# Autodesk Inventor assembly: ForeArmAssembly
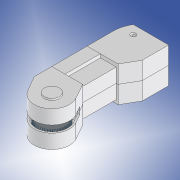
[picture p0: Inventor's stored thumbnail of the model, 180x180]
Saved by Autodesk Inventor 2017 (Build 210142000, 142)
## iProperties
Created: 2017-06-14
Part Number: ForeArmAssembly
Document SubType Name: Assembly
Designer: zallen
Author: zallen
## Documents named in this file (11)
- C:\Users\zallen\Documents\GitHub\cr-laundry-robot\src\Body\Arm Assembly\Bicep Assembly\BicepAssembly.iam
- C:\Users\zallen\Documents\GitHub\cr-laundry-robot\src\Body\Arm Assembly\Bicep Assembly\BA001.ipt
- C:\Users\zallen\Documents\GitHub\cr-laundry-robot\src\Body\Arm Assembly\Bicep Assembly\BA002.ipt
- C:\Users\zallen\Documents\GitHub\cr-laundry-robot\lib\Stepper Motor - NEMA 17\NEMA17.ipt
- C:\Users\zallen\Documents\GitHub\cr-laundry-robot\src\Body\Arm Assembly\Bicep Assembly\BA003.ipt
- C:\Users\zallen\Documents\GitHub\cr-laundry-robot\src\Body\Arm Assembly\Bicep Assembly\BA004.ipt
- C:\Users\zallen\Documents\GitHub\cr-laundry-robot\src\Body\Arm Assembly\Bicep Assembly\BA005.ipt
- C:\Users\zallen\Documents\GitHub\cr-laundry-robot\src\Body\Arm Assembly\Bicep Assembly\12 x 100mm Shaft.ipt
- C:\Users\zallen\Documents\GitHub\cr-laundry-robot\src\Body\Arm Assembly\Bicep Assembly\BicepAssembly\Design Accelerator\Spur Gears1.iam
- C:\Users\zallen\Documents\GitHub\cr-laundry-robot\lib\6201RS\6201RS.ipt
- C:\Users\zallen\Documents\GitHub\cr-laundry-robot\src\Body\Arm Assembly\Bicep Assembly\BA006.ipt
## Components (11 placed, 10 different names)
1. BA001:1 — Mate:1, Mate:3, Mate:4, Mate:5, Mate:8, Mate:12, Mate:18, Mate:41
2. BA002:1 — Mate:1, Mate:4, Mate:10, Mate:11
3. NEMA17:1 — Mate:3, Mate:5, Mate:18, Mate:40
4. BA003:1 — Mate:8, Mate:12, Mate:16, Mate:17
5. BA003:2 — Mate:10, Mate:11, Mate:13, Mate:14
6. BA004:1 — Mate:13, Mate:14, Mate:43, Mate:44
7. BA005:1 — Mate:16, Mate:17, Mate:19, Mate:20, Mate:33, Mate:38, Mate:42, Mate:43
8. 12 x 100mm Shaft:1 — Mate:19, Mate:20, Mate:35, Mate:44
9. Spur Gears:1 [sub-assembly] — Mate:33, Mate:35, Mate:36, Mate:37, Mate:38, Mate:42
10. 6201RS:1 — Mate:36, Mate:37
11. BA006:1 — Mate:40, Mate:41
## Relationships (25: Mate 25)
- Mate:1: BA001:1 ↔ BA002:1
- Mate:3: BA001:1 ↔ NEMA17:1
- Mate:4: BA001:1 ↔ BA002:1
- Mate:5: BA001:1 ↔ NEMA17:1
- Mate:8: BA001:1 ↔ BA003:1
- Mate:10: BA002:1 ↔ BA003:2
- Mate:11: BA002:1 ↔ BA003:2
- Mate:12: BA001:1 ↔ BA003:1
- Mate:13: BA003:2 ↔ BA004:1
- Mate:14: BA003:2 ↔ BA004:1
- Mate:16: BA003:1 ↔ BA005:1
- Mate:17: BA003:1 ↔ BA005:1
- Mate:18: BA001:1 ↔ NEMA17:1
- Mate:19: BA005:1 ↔ 12 x 100mm Shaft:1
- Mate:20: BA005:1 ↔ 12 x 100mm Shaft:1
- Mate:33: BA005:1 ↔ Spur Gears:1
- Mate:35: 12 x 100mm Shaft:1 ↔ Spur Gears:1
- Mate:36: Spur Gears:1 ↔ 6201RS:1
- Mate:37: Spur Gears:1 ↔ 6201RS:1
- Mate:38: BA005:1 ↔ Spur Gears:1
- Mate:40: NEMA17:1 ↔ BA006:1
- Mate:41: BA001:1 ↔ BA006:1
- Mate:42: BA005:1 ↔ Spur Gears:1
- Mate:43: BA004:1 ↔ BA005:1
- Mate:44: BA004:1 ↔ 12 x 100mm Shaft:1
